# Autodesk Inventor assembly: Ultibots200x250Bed
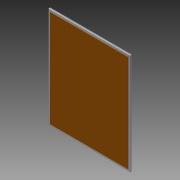
[picture p0: Inventor's stored thumbnail of the model, 180x180]
Saved by Autodesk Inventor 2015 (Build 190159000, 159)
## iProperties
Created: 2014-10-10
Part Number: Ultibots200x250Bed
Document SubType Name: Assembly
Designer: Jack
Author: Jack
## Documents named in this file (4)
- C:\Users\Jack\ownCloud\Projects\CoreXY\InventorModel\HeatBed\Ultibots200x250\Ultibots200x250Bed.iam
- C:\Users\Jack\ownCloud\Projects\CoreXY\InventorModel\HeatBed\Ultibots200x250\Ultibots200x250KaptonHeater.ipt
- C:\Users\Jack\ownCloud\Projects\CoreXY\InventorModel\HeatBed\Ultibots200x250\Ultibots200x250HeatSpreader.ipt
- C:\Users\Jack\ownCloud\Projects\CoreXY\InventorModel\HeatBed\Ultibots200x250\Ultibots200x250Glass.ipt
## Components (3 placed, 3 different names)
1. Ultibots200x250KaptonHeater:1 — Mate:1, Flush:1, Flush:2, Mate:2, Flush:5, Flush:6
2. Ultibots200x250HeatSpreader:1 — Mate:2, Mate:3, Flush:3, Flush:4, Flush:5
3. Ultibots200x250Glass:1 — Mate:3, Flush:3, Flush:4, Flush:6
## Relationships (9: Flush 6, Mate 3)
- Mate:1: Ultibots200x250KaptonHeater:1
- Flush:1: Ultibots200x250KaptonHeater:1
- Flush:2: Ultibots200x250KaptonHeater:1
- Mate:2: Ultibots200x250KaptonHeater:1 ↔ Ultibots200x250HeatSpreader:1
- Mate:3: Ultibots200x250HeatSpreader:1 ↔ Ultibots200x250Glass:1
- Flush:3: Ultibots200x250HeatSpreader:1 ↔ Ultibots200x250Glass:1
- Flush:4: Ultibots200x250HeatSpreader:1 ↔ Ultibots200x250Glass:1
- Flush:5 (-5 mm): Ultibots200x250KaptonHeater:1 ↔ Ultibots200x250HeatSpreader:1
- Flush:6 (-5 mm): Ultibots200x250KaptonHeater:1 ↔ Ultibots200x250Glass:1
